# Autodesk Inventor assembly: Spinn105_Subrack
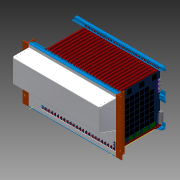
[picture p0: Inventor's stored thumbnail of the model, 180x180]
Saved by Autodesk Inventor 2015 SP1 (Build 190203100, 203)
## iProperties
Created: 2014-08-23
Part Number: Spinn105_Subrack
Document SubType Name: Assembly
Designer: Patrick Camilleri
Author: Patrick Camilleri
## Documents named in this file (8)
- C:\Users\Patrick\EDA\CAD\Spin5 Subrack\Spinn105_Subrack.iam
- C:\Users\Patrick\EDA\CAD\Spin5 Subrack\GuideRail_24560353.ipt
- C:\Users\Patrick\EDA\CAD\Spin5 Subrack\Imported Components\24563492\24563492.iam
- C:\Users\Patrick\EDA\CAD\Spin5 Board\Spin5 Inventor nores nocap\Imported Components\spin5v1_simple_2\spin5v1_simple_2.iam
- C:\Users\Patrick\EDA\CAD\Spin5 Subrack\subrack_frontpanel.ipt
- C:\Users\Patrick\EDA\CAD\Sata Shielding\Shield.ipt
- C:\Users\Patrick\EDA\CAD\Sata Shielding\Shield_noflanges.ipt
- C:\Users\Patrick\EDA\CAD\Sata Shielding\Shield_noflanges2.ipt
## Components (77 placed, 7 different names)
1. 24563492:1 [sub-assembly] — Rigid:3, Rigid:4, Mate:3, Mate:4, Mate:5, Mate:8, Mate:11
2. subrack_frontpanel:1
3. Shield:1 — Mate:3, Mate:6, Mate:7
4. Shield_noflanges:1 — Mate:8, Mate:9, Mate:10
5. Shield_noflanges2:1 — Mate:11, Mate:12, Mate:13
6. GuideRail_24560353:1 — Rigid:3, Rigid:5
7. GuideRail_24560353:3
8. GuideRail_24560353:4
9. GuideRail_24560353:5
10. GuideRail_24560353:6
11. GuideRail_24560353:7
12. GuideRail_24560353:8
13. GuideRail_24560353:9
14. GuideRail_24560353:10
15. GuideRail_24560353:11
16. GuideRail_24560353:12
17. GuideRail_24560353:13
18. GuideRail_24560353:14
19. GuideRail_24560353:15
20. GuideRail_24560353:16
21. GuideRail_24560353:17
22. GuideRail_24560353:18
23. GuideRail_24560353:19
24. GuideRail_24560353:20
25. GuideRail_24560353:21
26. GuideRail_24560353:22
27. GuideRail_24560353:23
28. GuideRail_24560353:24
29. GuideRail_24560353:25
30. GuideRail_24560353:2 — Rigid:4
31. GuideRail_24560353:26
32. GuideRail_24560353:27
33. GuideRail_24560353:28
34. GuideRail_24560353:29
35. GuideRail_24560353:30
36. GuideRail_24560353:31
37. GuideRail_24560353:32
38. GuideRail_24560353:33
39. GuideRail_24560353:34
40. GuideRail_24560353:35
41. GuideRail_24560353:36
42. GuideRail_24560353:37
43. GuideRail_24560353:38
44. GuideRail_24560353:39
45. GuideRail_24560353:40
46. GuideRail_24560353:41
47. GuideRail_24560353:42
48. GuideRail_24560353:43
49. GuideRail_24560353:44
50. GuideRail_24560353:45
51. GuideRail_24560353:46
52. GuideRail_24560353:47
53. GuideRail_24560353:48
54. spin5v1_simple_2:1 [sub-assembly] — Rigid:5
55. spin5v1_simple_2:2 [sub-assembly]
56. spin5v1_simple_2:3 [sub-assembly]
57. spin5v1_simple_2:4 [sub-assembly]
58. spin5v1_simple_2:5 [sub-assembly]
59. spin5v1_simple_2:6 [sub-assembly]
60. spin5v1_simple_2:7 [sub-assembly]
61. spin5v1_simple_2:8 [sub-assembly]
62. spin5v1_simple_2:9 [sub-assembly]
63. spin5v1_simple_2:10 [sub-assembly]
64. spin5v1_simple_2:11 [sub-assembly]
65. spin5v1_simple_2:12 [sub-assembly]
66. spin5v1_simple_2:13 [sub-assembly]
67. spin5v1_simple_2:14 [sub-assembly]
68. spin5v1_simple_2:15 [sub-assembly]
69. spin5v1_simple_2:16 [sub-assembly]
70. spin5v1_simple_2:17 [sub-assembly]
71. spin5v1_simple_2:18 [sub-assembly]
72. spin5v1_simple_2:19 [sub-assembly]
73. spin5v1_simple_2:20 [sub-assembly]
74. spin5v1_simple_2:21 [sub-assembly]
75. spin5v1_simple_2:22 [sub-assembly]
76. spin5v1_simple_2:23 [sub-assembly]
77. spin5v1_simple_2:24 [sub-assembly]
## Component patterns: (24 elements, first: GuideRail_24560353:1), (24 elements, first: GuideRail_24560353:2), (24 elements, first: spin5v1_simple_2:1)
## Relationships (14: Mate 11, WeldJoint 3)
- Rigid:3 [WeldJoint]: 24563492:1 ↔ GuideRail_24560353:1
- Rigid:4 [WeldJoint]: 24563492:1 ↔ GuideRail_24560353:2
- Rigid:5 [WeldJoint]: GuideRail_24560353:1 ↔ spin5v1_simple_2:1
- Mate:3: 24563492:1 ↔ Shield:1
- Mate:4: 24563492:1
- Mate:5: 24563492:1
- Mate:6: Shield:1
- Mate:7: Shield:1
- Mate:8: 24563492:1 ↔ Shield_noflanges:1
- Mate:9: Shield_noflanges:1
- Mate:10: Shield_noflanges:1
- Mate:11: 24563492:1 ↔ Shield_noflanges2:1
- Mate:12: Shield_noflanges2:1
- Mate:13: Shield_noflanges2:1
